# Autodesk Inventor assembly: TireSensorCase_Assembly
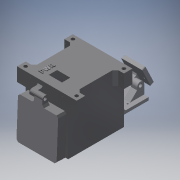
[picture p0: Inventor's stored thumbnail of the model, 180x180]
Saved by Autodesk Inventor 2018 (Build 220112000, 112)
## iProperties
Created: 2020-10-25
Part Number: TireSensorCase_Assembly
Document SubType Name: Assembly
Designer: tbrow
Author: tbrow
## Documents named in this file (5)
- C:\Users\tbrow\OneDrive\Documents\Arduino1.8.5\Maple-Mini-Kart-Daq\CaseCAD\TireSensorCase\TireSensorCase_Assembly.iam
- C:\Users\tbrow\OneDrive\Documents\Arduino1.8.5\Maple-Mini-Kart-Daq\CaseCAD\TireSensorCase\TireSensorCase_Main.ipt
- C:\Users\tbrow\OneDrive\Documents\Arduino1.8.5\Maple-Mini-Kart-Daq\CaseCAD\TireSensorCase\TireSensorCase_TopCover.ipt
- C:\Users\tbrow\OneDrive\Documents\Arduino1.8.5\Maple-Mini-Kart-Daq\CaseCAD\Mount for TMP007 Sensor.ipt
- C:\Users\tbrow\OneDrive\Documents\Arduino1.8.5\Maple-Mini-Kart-Daq\CaseCAD\MMandBatteryCover.ipt
## Components (4 placed, 4 different names)
1. TireSensorCase_Main:1 — Mate:1, Angle:1, Insert:1, Insert:2
2. TireSensorCase_TopCover:1 — Mate:1, Angle:1
3. Mount for TMP007 Sensor:1 — Insert:1
4. MMandBatteryCover:1 — Insert:2
## Relationships (4: Insert 2, Mate 1, Angle 1)
- Mate:1: TireSensorCase_Main:1 ↔ TireSensorCase_TopCover:1
- Angle:1 (0 deg): TireSensorCase_Main:1 ↔ TireSensorCase_TopCover:1
- Insert:1: TireSensorCase_Main:1 ↔ Mount for TMP007 Sensor:1
- Insert:2: TireSensorCase_Main:1 ↔ MMandBatteryCover:1
